# Autodesk Inventor assembly: foiurbar_MIR
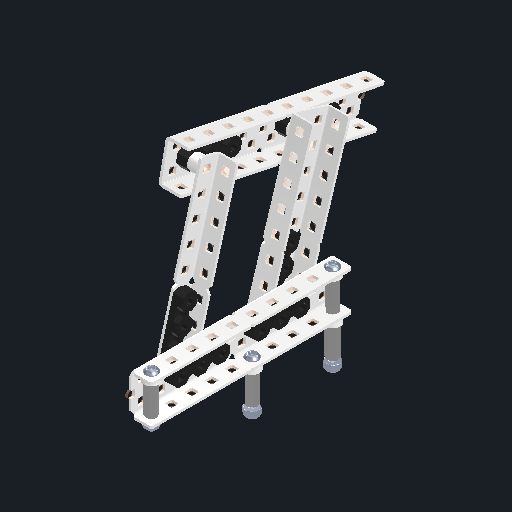
[picture p0: Inventor's stored thumbnail of the model, 512x512]
Saved by Autodesk Inventor 2023 (Build 270158000, 158)
## iProperties
Created: 2023-08-08
Part Number: foiurbar_MIR
Document SubType Name: Assembly
Designer: srbel
Author: srbel
## Documents named in this file (14)
- C:\CAD\OverUnderCAD\Drive\foiurbar_MIR.iam
- C:\CAD\OverUnderCAD\VEX-CAD-Inventor-1.4.0\Structure\C Channel\Aluminum 1x2x1\Alu C 1x2x1x10_MIR.ipt
- C:\CAD\OverUnderCAD\VEX-CAD-Inventor-1.4.0\Motion\Spacers\Spacer Nylon .313 OD\NSpacer .313 OD x .125.ipt
- C:\CAD\OverUnderCAD\VEX-CAD-Inventor-1.4.0\Motion\Spacers\Spacer Nylon .313 OD.ipt
- C:\CAD\OverUnderCAD\VEX-CAD-Inventor-1.4.0\Structure\Standoff\Standoff .75.ipt
- C:\CAD\OverUnderCAD\VEX-CAD-Inventor-1.4.0\Structure\Standoff.ipt
- C:\CAD\OverUnderCAD\VEX-CAD-Inventor-1.4.0\Structure\Hardware\Screw Steel - Star\SScrew Star Threaded 2.250.ipt
- C:\CAD\OverUnderCAD\VEX-CAD-Inventor-1.4.0\Structure\Hardware\Screw Steel - Star.ipt
- C:\CAD\OverUnderCAD\VEX-CAD-Inventor-1.4.0\Structure\Hardware\Nut Thin Nylock_MIR6.ipt
- C:\CAD\OverUnderCAD\VEX-CAD-Inventor-1.4.0\Structure\Hardware\Screw Steel - Star\SScrew Star Threaded 1.250.ipt
- C:\CAD\OverUnderCAD\VEX-CAD-Inventor-1.4.0\Motion\Shaft LS\Bearing Flat_MIR1.ipt
- C:\CAD\OverUnderCAD\VEX-CAD-Inventor-1.4.0\Structure\Angle\Aluminum\1x1\Alu Angle 1x1x8_MIR.ipt
- C:\CAD\OverUnderCAD\VEX-CAD-Inventor-1.4.0\Structure\C Channel\Aluminum 1x2x1\Alu C 1x2x1x8_MIR.ipt
- C:\CAD\OverUnderCAD\VEX-CAD-Inventor-1.4.0\Motion\Spacers\Spacer Nylon .313 OD\NSpacer .313 OD x .250.ipt
## Components (28 placed, 10 different names)
1. Alu C 1x2x1x10_MIR:1 — Insert:2, Insert:4, Insert:6, Insert:7, Insert:10, Insert:11, Insert:16, Insert:18, Insert:17, Insert:19, Insert:20, Insert:62, Insert:63
2. NSpacer .313 OD x .125:1 — Insert:2, Insert:1
3. Standoff .75:1 — Insert:1
4. NSpacer .313 OD x .125:2 — Insert:4, Insert:3
5. Standoff .75:2 — Insert:3
6. Standoff .75:3 — Insert:8, Insert:15
7. NSpacer .313 OD x .125:3 — Insert:6, Insert:5
8. Standoff .75:4 — Insert:5, Insert:9
9. SScrew Star Threaded 2.250:1 — Insert:7
10. Nut Thin Nylock_MIR6:1 — Insert:9
11. Nut Thin Nylock_MIR6:2 — Insert:8
12. Nut Thin Nylock_MIR6:3 — Insert:10
13. SScrew Star Threaded 1.250:2 — Insert:11
14. NSpacer .313 OD x .125:4 — Insert:16, Insert:15
15. Bearing Flat_MIR1:1 — Insert:18, Insert:17
16. Bearing Flat_MIR1:2 — Insert:19
17. SScrew Star Threaded 1.250:3 — Insert:20
18. Bearing Flat_MIR1:3 — Insert:55, Insert:54, Insert:60
19. Bearing Flat_MIR1:4 — Insert:53, Insert:52, Insert:61
20. Alu Angle 1x1x8_MIR:1 — Insert:53, Insert:52, Insert:65
21. Alu C 1x2x1x8_MIR:1 — Insert:55, Insert:54, Insert:69
22. Alu C 1x2x1x10_MIR:2 — Insert:57, Insert:56, Insert:68, Insert:67
23. Bearing Flat_MIR1:5 — Insert:57, Insert:56, Insert:64
24. NSpacer .313 OD x .250:5 — Insert:62, Insert:60
25. NSpacer .313 OD x .250:6 — Insert:63, Insert:61
26. NSpacer .313 OD x .250:7 — Insert:65, Insert:64
27. Bearing Flat_MIR1:6 — Insert:68, Insert:67, Insert:66
28. NSpacer .313 OD x .250:8 — Insert:69, Insert:66
## Relationships (33: Insert 33)
- Insert:2: Alu C 1x2x1x10_MIR:1 ↔ NSpacer .313 OD x .125:1
- Insert:1: NSpacer .313 OD x .125:1 ↔ Standoff .75:1
- Insert:4: Alu C 1x2x1x10_MIR:1 ↔ NSpacer .313 OD x .125:2
- Insert:3: NSpacer .313 OD x .125:2 ↔ Standoff .75:2
- Insert:6 (1.5875 mm): Alu C 1x2x1x10_MIR:1 ↔ NSpacer .313 OD x .125:3
- Insert:5: NSpacer .313 OD x .125:3 ↔ Standoff .75:4
- Insert:7: Alu C 1x2x1x10_MIR:1 ↔ SScrew Star Threaded 2.250:1
- Insert:9 (1.5875 mm): Standoff .75:4 ↔ Nut Thin Nylock_MIR6:1
- Insert:8 (1.5875 mm): Standoff .75:3 ↔ Nut Thin Nylock_MIR6:2
- Insert:10: Alu C 1x2x1x10_MIR:1 ↔ Nut Thin Nylock_MIR6:3
- Insert:11: Alu C 1x2x1x10_MIR:1 ↔ SScrew Star Threaded 1.250:2
- Insert:16 (1.5875 mm): Alu C 1x2x1x10_MIR:1 ↔ NSpacer .313 OD x .125:4
- Insert:15: Standoff .75:3 ↔ NSpacer .313 OD x .125:4
- Insert:18: Alu C 1x2x1x10_MIR:1 ↔ Bearing Flat_MIR1:1
- Insert:17: Alu C 1x2x1x10_MIR:1 ↔ Bearing Flat_MIR1:1
- Insert:19: Alu C 1x2x1x10_MIR:1 ↔ Bearing Flat_MIR1:2
- Insert:20: Alu C 1x2x1x10_MIR:1 ↔ SScrew Star Threaded 1.250:3
- Insert:53: Bearing Flat_MIR1:4 ↔ Alu Angle 1x1x8_MIR:1
- Insert:52: Bearing Flat_MIR1:4 ↔ Alu Angle 1x1x8_MIR:1
- Insert:55: Bearing Flat_MIR1:3 ↔ Alu C 1x2x1x8_MIR:1
- Insert:54: Bearing Flat_MIR1:3 ↔ Alu C 1x2x1x8_MIR:1
- Insert:57: Alu C 1x2x1x10_MIR:2 ↔ Bearing Flat_MIR1:5
- Insert:56: Alu C 1x2x1x10_MIR:2 ↔ Bearing Flat_MIR1:5
- Insert:62: Alu C 1x2x1x10_MIR:1 ↔ NSpacer .313 OD x .250:5
- Insert:60: Bearing Flat_MIR1:3 ↔ NSpacer .313 OD x .250:5
- Insert:63: Alu C 1x2x1x10_MIR:1 ↔ NSpacer .313 OD x .250:6
- Insert:61: Bearing Flat_MIR1:4 ↔ NSpacer .313 OD x .250:6
- Insert:65: Alu Angle 1x1x8_MIR:1 ↔ NSpacer .313 OD x .250:7
- Insert:64: Bearing Flat_MIR1:5 ↔ NSpacer .313 OD x .250:7
- Insert:68: Alu C 1x2x1x10_MIR:2 ↔ Bearing Flat_MIR1:6
- Insert:67: Alu C 1x2x1x10_MIR:2 ↔ Bearing Flat_MIR1:6
- Insert:69: Alu C 1x2x1x8_MIR:1 ↔ NSpacer .313 OD x .250:8
- Insert:66: Bearing Flat_MIR1:6 ↔ NSpacer .313 OD x .250:8
